# Autodesk Inventor assembly: aseembly
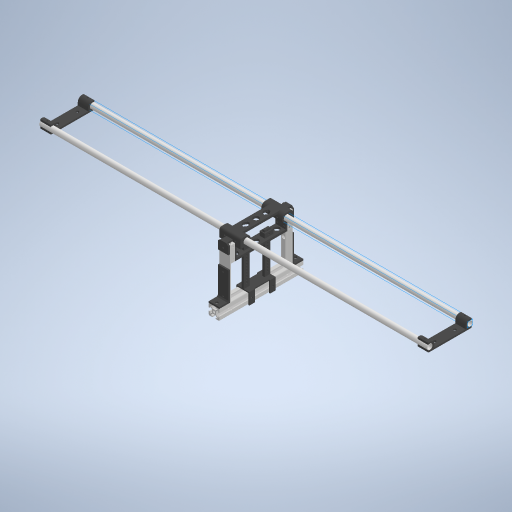
[picture p0: Inventor's stored thumbnail of the model, 512x512]
Saved by Autodesk Inventor 2024.3 (Build 283343000, 343)
## iProperties
Created: 2024-09-08
Part Number: aseembly
Document SubType Name: Assembly
Designer: Gihyeok
Author: Gihyeok
## Documents named in this file (9)
- C:\Users\gihyeok2\Desktop\New folder\component\linear_guide\dummy_assembly.iam
- C:\Users\gihyeok2\Desktop\New folder\component\linear_guide\HFS5-2020-160-AH24-BH136-Z6-XA20-XB65-XC140_Autodesk_Inventor_2024_20240908\HFS5-2020-160-AH24-BH136-Z6-XA20-XB65-XC140.ipt
- C:\Users\gihyeok2\Desktop\New folder\component\linear_guide\base.ipt
- C:\Users\gihyeok2\Desktop\New folder\component\linear_guide\linear_rail(JKSG10-95-S1)\JKSG10-95-S1.iam
- C:\Users\gihyeok2\Desktop\New folder\component\linear_guide\top.ipt
- C:\Users\gihyeok2\Desktop\New folder\component\linear_guide\pillar_2ea.ipt
- C:\Users\gihyeok2\Desktop\New folder\component\linear_guide\latch.ipt
- D:\OneDrive\Tokyo Tech\Project\Dog Robot\Hoshiramu_robot\component\linear_guide\aluminium_pipe_10mm_740mm.ipt
- C:\Users\gihyeok2\Desktop\New folder\component\linear_guide\pipe_holder.ipt
## Components (13 placed, 8 different names)
1. HFS5-2020-160-AH24-BH136-Z6-XA20-XB65-XC140:1 — Mate:17, Mate:18, Flush:2, Mate:19, Mate:20
2. base:1 — Mate:14, Mate:15, Mate:16
3. base:2 — Mate:11, Mate:12, Mate:13, Mate:17, Mate:18, Flush:2
4. JKSG10-95-S1:2 [sub-assembly] — Mate:1, Mate:2, Mate:6, Mate:9, Mate:10, Flush:1, Mate:14, Mate:15, Mate:16
5. top:1 — Mate:1, Mate:2, Mate:3, Mate:4, Mate:5, Mate:6, Mate:21, Mate:22, Mate:23, Mate:24, Mate:25
6. JKSG10-95-S1:3 [sub-assembly] — Mate:3, Mate:4, Mate:5, Mate:7, Mate:8, Mate:11, Mate:12, Mate:13
7. pillar_2ea:1 — Mate:19, Mate:20, Mate:21
8. latch:1 — Mate:7, Mate:8
9. latch:2 — Mate:9, Mate:10, Flush:1
10. aluminium_pipe_10mm_740mm:1 — Mate:22, Mate:23, Mate:28, Mate:29
11. aluminium_pipe_10mm_740mm:2 — Mate:24, Mate:25, Mate:26, Mate:27
12. pipe_holder:1 — Mate:26, Mate:27
13. pipe_holder:2 — Mate:28, Mate:29
## Relationships (31: Mate 29, Flush 2)
- Mate:1: JKSG10-95-S1:2 ↔ top:1
- Mate:2: JKSG10-95-S1:2 ↔ top:1
- Mate:3: top:1 ↔ JKSG10-95-S1:3
- Mate:4: top:1 ↔ JKSG10-95-S1:3
- Mate:5: top:1 ↔ JKSG10-95-S1:3
- Mate:6: JKSG10-95-S1:2 ↔ top:1
- Mate:7: JKSG10-95-S1:3 ↔ latch:1
- Mate:8: JKSG10-95-S1:3 ↔ latch:1
- Mate:9: JKSG10-95-S1:2 ↔ latch:2
- Mate:10: JKSG10-95-S1:2 ↔ latch:2
- Flush:1: JKSG10-95-S1:2 ↔ latch:2
- Mate:11: base:2 ↔ JKSG10-95-S1:3
- Mate:12: base:2 ↔ JKSG10-95-S1:3
- Mate:13: base:2 ↔ JKSG10-95-S1:3
- Mate:14: base:1 ↔ JKSG10-95-S1:2
- Mate:15: base:1 ↔ JKSG10-95-S1:2
- Mate:16: base:1 ↔ JKSG10-95-S1:2
- Mate:17: HFS5-2020-160-AH24-BH136-Z6-XA20-XB65-XC140:1 ↔ base:2
- Mate:18: HFS5-2020-160-AH24-BH136-Z6-XA20-XB65-XC140:1 ↔ base:2
- Flush:2: HFS5-2020-160-AH24-BH136-Z6-XA20-XB65-XC140:1 ↔ base:2
- Mate:19: HFS5-2020-160-AH24-BH136-Z6-XA20-XB65-XC140:1 ↔ pillar_2ea:1
- Mate:20: HFS5-2020-160-AH24-BH136-Z6-XA20-XB65-XC140:1 ↔ pillar_2ea:1
- Mate:21: top:1 ↔ pillar_2ea:1
- Mate:22: top:1 ↔ aluminium_pipe_10mm_740mm:1
- Mate:23: top:1 ↔ aluminium_pipe_10mm_740mm:1
- Mate:24: top:1 ↔ aluminium_pipe_10mm_740mm:2
- Mate:25: top:1 ↔ aluminium_pipe_10mm_740mm:2
- Mate:26: aluminium_pipe_10mm_740mm:2 ↔ pipe_holder:1
- Mate:27: aluminium_pipe_10mm_740mm:2 ↔ pipe_holder:1
- Mate:28: aluminium_pipe_10mm_740mm:1 ↔ pipe_holder:2
- Mate:29: aluminium_pipe_10mm_740mm:1 ↔ pipe_holder:2
